# Autodesk Inventor assembly: FE-120 Door Section
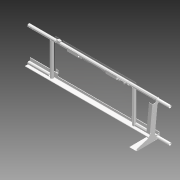
[picture p0: Inventor's stored thumbnail of the model, 180x180]
Saved by Autodesk Inventor 2021 (Build 250183000, 183)
## iProperties
Created: 2021-01-11
Part Number: FE-120 Door Section
Document SubType Name: Assembly
## Documents named in this file (15)
- D:\FIRST\Design\FRC Fields\Generic Field Base\FE-100 Side Wall\FE-120 Door Section\FE-120 Door Section.iam
- D:\FIRST\Design\FRC Fields\Generic Field Base\FE-100 Side Wall\FE-110 Main Section\FE-110-004 Bottom Side Bar.ipt
- D:\FIRST\Design\FRC Fields\Generic Field Base\FE-100 Side Wall\FE-110 Main Section\FE-110-006 Side Holder.ipt
- D:\FIRST\Design\FRC Fields\Generic Field Base\FE-100 Side Wall\FE-120 Door Section\FE-120-001 Floor L Section.ipt
- D:\FIRST\Design\FRC Fields\Generic Field Base\FE-100 Side Wall\FE-120 Door Section\FE-120-002 Top Connector Bar.ipt
- D:\FIRST\Design\FRC Fields\Generic Field Base\FE-100 Side Wall\FE-120 Door Section\FE-120-003 Upright Middle Section.ipt
- D:\FIRST\Design\FRC Fields\Generic Field Base\FE-100 Side Wall\FE-120 Door Section\FE-120-004 Pivot Hardstop.ipt
- D:\FIRST\Design\FRC Fields\Generic Field Base\FE-100 Side Wall\FE-110 Main Section\FE-110-005 Inside Connector Bar.ipt
- D:\FIRST\Design\FRC Fields\Generic Field Base\FE-100 Side Wall\FE-120 Door Section\FE-120-005 Door Insert.ipt
- D:\FIRST\Design\FRC Fields\Generic Field Base\FE-100 Side Wall\FE-120 Door Section\FE-120-006 Hinge.ipt
- D:\FIRST\Design\FRC Fields\Generic Field Base\FE-100 Side Wall\FE-120 Door Section\FE-120-007 Door Tube.ipt
- D:\FIRST\Design\FRC Fields\Generic Field Base\FE-100 Side Wall\FE-120 Door Section\FE-120-008 Pin.ipt
- D:\FIRST\Design\FRC Fields\Generic Field Base\FE-100 Side Wall\FE-120 Door Section\FE-120-009 Door Panel.ipt
- D:\FIRST\Design\FRC Fields\Generic Field Base\FE-100 Side Wall\FE-120 Door Section\FE-120-010 Tube Holder.ipt
- D:\FIRST\Design\FRC Fields\Generic Field Base\FE-100 Side Wall\FE-120 Door Section\FE-120-011 Bottom Bent Piece.ipt
## Components (21 placed, 14 different names)
1. FE-120-001 Floor L Section:1 — Tangent:2, Flush:2, Tangent:3, Flush:4, Angle:1, Mate:3, Mate:5, Flush:11, Angle:2, Mate:19, Flush:13
2. FE-110-004 Bottom Side Bar:1 — Tangent:2, Flush:2, Tangent:4, Mate:2, Flush:8, Mate:6, Mate:10, Mate:12, Mate:13
3. FE-110-004 Bottom Side Bar:2 — Tangent:3, Flush:4, Flush:6, Mate:2, Flush:7, Angle:1, Mate:3, Mate:4, Mate:7, Mate:13
4. FE-110-006 Side Holder:1 — Tangent:4, Insert:1
5. FE-120-002 Top Connector Bar:1 — Mate:1, Flush:5, Flush:6, Flush:7, Mate:4, Mate:14, Mate:15, Tangent:6
6. FE-120-002 Top Connector Bar:2 — Mate:1, Flush:5, Flush:8, Insert:1, Flush:12, Mate:8, Mate:9, Mate:11, Insert:2
7. FE-120-003 Upright Middle Section:1 — Flush:9, Flush:10, Mate:5, Flush:11, Mate:6
8. FE-120-003 Upright Middle Section:2 — Flush:9, Flush:10, Mate:7
9. FE-120-004 Pivot Hardstop:1 — Flush:12, Mate:8, Angle:2
10. FE-110-005 Inside Connector Bar:1 — Mate:9, Mate:11
11. FE-110-005 Inside Connector Bar:2 — Mate:10, Mate:12
12. FE-120-005 Door Insert:1 — Insert:2, Angle:3, Mate:16, Mate:17, Mate:18
13. FE-120-006 Hinge:1 — Insert:3
14. FE-120-006 Hinge:2 — Mate:14, Mate:15, Insert:3
15. FE-120-007 Door Tube:1 — Mate:16, Mate:17, Tangent:5
16. FE-120-008 Pin:1 — Mate:18, Tangent:5
17. FE-120-009 Door Panel:1 — Mate:19, Flush:13, Tangent:6, Insert:4, Insert:5, Insert:6, Insert:7, Insert:8, Insert:9, Insert:10, Insert:11
18. FE-120-010 Tube Holder:1 — Insert:4, Insert:5
19. FE-120-010 Tube Holder:2 — Insert:6, Insert:7
20. FE-120-011 Bottom Bent Piece:1 — Insert:8, Insert:9
21. FE-120-011 Bottom Bent Piece:2 — Insert:10, Insert:11
## Relationships (49: Mate 19, Flush 11, Insert 11, Tangent 5, Angle 3)
- Tangent:2: FE-120-001 Floor L Section:1 ↔ FE-110-004 Bottom Side Bar:1
- Flush:2 (6.35 mm): FE-120-001 Floor L Section:1 ↔ FE-110-004 Bottom Side Bar:1
- Tangent:3: FE-120-001 Floor L Section:1 ↔ FE-110-004 Bottom Side Bar:2
- Flush:4 (6.35 mm): FE-120-001 Floor L Section:1 ↔ FE-110-004 Bottom Side Bar:2
- Tangent:4: FE-110-004 Bottom Side Bar:1 ↔ FE-110-006 Side Holder:1
- Mate:1: FE-120-002 Top Connector Bar:1 ↔ FE-120-002 Top Connector Bar:2
- Flush:5: FE-120-002 Top Connector Bar:1 ↔ FE-120-002 Top Connector Bar:2
- Flush:6: FE-110-004 Bottom Side Bar:2 ↔ FE-120-002 Top Connector Bar:1
- Mate:2: FE-110-004 Bottom Side Bar:1 ↔ FE-110-004 Bottom Side Bar:2
- Flush:7: FE-110-004 Bottom Side Bar:2 ↔ FE-120-002 Top Connector Bar:1
- Flush:8: FE-110-004 Bottom Side Bar:1 ↔ FE-120-002 Top Connector Bar:2
- Angle:1 (0 deg): FE-120-001 Floor L Section:1 ↔ FE-110-004 Bottom Side Bar:2
- Mate:3 (21.082 mm): FE-120-001 Floor L Section:1 ↔ FE-110-004 Bottom Side Bar:2
- Mate:4 (459.1749 mm): FE-110-004 Bottom Side Bar:2 ↔ FE-120-002 Top Connector Bar:1
- Insert:1: FE-110-006 Side Holder:1 ↔ FE-120-002 Top Connector Bar:2
- Flush:9: FE-120-003 Upright Middle Section:1 ↔ FE-120-003 Upright Middle Section:2
- Flush:10: FE-120-003 Upright Middle Section:1 ↔ FE-120-003 Upright Middle Section:2
- Mate:5: FE-120-001 Floor L Section:1 ↔ FE-120-003 Upright Middle Section:1
- Flush:11 (-21.082 mm): FE-120-001 Floor L Section:1 ↔ FE-120-003 Upright Middle Section:1
- Mate:6 (24.6126 mm): FE-110-004 Bottom Side Bar:1 ↔ FE-120-003 Upright Middle Section:1
- Mate:7 (24.6126 mm): FE-110-004 Bottom Side Bar:2 ↔ FE-120-003 Upright Middle Section:2
- Flush:12 (-12.7 mm): FE-120-002 Top Connector Bar:2 ↔ FE-120-004 Pivot Hardstop:1
- Mate:8: FE-120-002 Top Connector Bar:2 ↔ FE-120-004 Pivot Hardstop:1
- Angle:2 (0 deg): FE-120-001 Floor L Section:1 ↔ FE-120-004 Pivot Hardstop:1
- Mate:9: FE-120-002 Top Connector Bar:2 ↔ FE-110-005 Inside Connector Bar:1
- Mate:10: FE-110-004 Bottom Side Bar:1 ↔ FE-110-005 Inside Connector Bar:2
- Mate:11: FE-120-002 Top Connector Bar:2 ↔ FE-110-005 Inside Connector Bar:1
- Mate:12: FE-110-004 Bottom Side Bar:1 ↔ FE-110-005 Inside Connector Bar:2
- Mate:13: FE-110-004 Bottom Side Bar:1 ↔ FE-110-004 Bottom Side Bar:2
- Insert:2 (-117.475 mm): FE-120-002 Top Connector Bar:2 ↔ FE-120-005 Door Insert:1
- Angle:3 (0 deg): FE-120-005 Door Insert:1
- Mate:14: FE-120-002 Top Connector Bar:1 ↔ FE-120-006 Hinge:2
- Mate:15: FE-120-002 Top Connector Bar:1 ↔ FE-120-006 Hinge:2
- Insert:3: FE-120-006 Hinge:1 ↔ FE-120-006 Hinge:2
- Mate:16: FE-120-005 Door Insert:1 ↔ FE-120-007 Door Tube:1
- Mate:17: FE-120-005 Door Insert:1 ↔ FE-120-007 Door Tube:1
- Mate:18: FE-120-005 Door Insert:1 ↔ FE-120-008 Pin:1
- Tangent:5: FE-120-007 Door Tube:1 ↔ FE-120-008 Pin:1
- Mate:19: FE-120-001 Floor L Section:1 ↔ FE-120-009 Door Panel:1
- Flush:13: FE-120-001 Floor L Section:1 ↔ FE-120-009 Door Panel:1
- Tangent:6: FE-120-002 Top Connector Bar:1 ↔ FE-120-009 Door Panel:1
- Insert:4: FE-120-009 Door Panel:1 ↔ FE-120-010 Tube Holder:1
- Insert:5: FE-120-009 Door Panel:1 ↔ FE-120-010 Tube Holder:1
- Insert:6: FE-120-009 Door Panel:1 ↔ FE-120-010 Tube Holder:2
- Insert:7: FE-120-009 Door Panel:1 ↔ FE-120-010 Tube Holder:2
- Insert:8: FE-120-009 Door Panel:1 ↔ FE-120-011 Bottom Bent Piece:1
- Insert:9: FE-120-009 Door Panel:1 ↔ FE-120-011 Bottom Bent Piece:1
- Insert:10: FE-120-009 Door Panel:1 ↔ FE-120-011 Bottom Bent Piece:2
- Insert:11: FE-120-009 Door Panel:1 ↔ FE-120-011 Bottom Bent Piece:2
